# Autodesk Inventor assembly: Motor_25GA370-226x1-6V-21RPM_MIR1
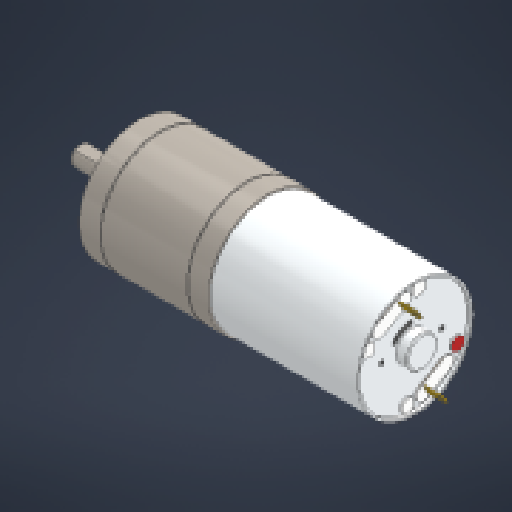
[picture p0: Inventor's stored thumbnail of the model, 512x512]
Saved by Autodesk Inventor 2026.1 (Build 301233000, 233)
## iProperties
Created: 2023-10-13
Part Number: Motor_25GA370-226x1-6V-21RPM_MIR1
Description: STEP AP214
Document SubType Name: Assembly
Designer: momen
Title: Motor_25GA370-226x1-6V-21RPM.STEP
Author: Wurs
Revision Number: ANY
Sending System: SolidWorks 2022
Preprocessor: SwSTEP 2.0
## Documents named in this file (3)
- D:\momen\Eng.-ASU\Senior1\MCT Sys design\design\old design\Motor_25GA370-226x1-6V-21RPM_MIR1.iam
- D:\momen\Eng.-ASU\Senior1\MCT Sys design\design\old design\Motor_25GA370-226x_MIR1.ipt
- D:\momen\Eng.-ASU\Senior1\MCT Sys design\design\old design\pan cross head_am_B18.6.7M - M2.5 x 0.45 x 3 Type I Cross Recessed PHMS --3N_MIR1.ipt
## Components (3 placed, 2 different names)
1. Motor_25GA370-226x_MIR1:1 — Tangent:1
2. pan cross head_am_B18.6.7M - M2.5 x 0.45 x 3 Type I Cross Recessed PHMS --3N_MIR1:1
3. pan cross head_am_B18.6.7M - M2.5 x 0.45 x 3 Type I Cross Recessed PHMS --3N_MIR1:2
## Relationships (1: Tangent 1)
- Tangent:1: Motor_25GA370-226x_MIR1:1
